# Autodesk Inventor assembly: Ball-Balancing-Robot
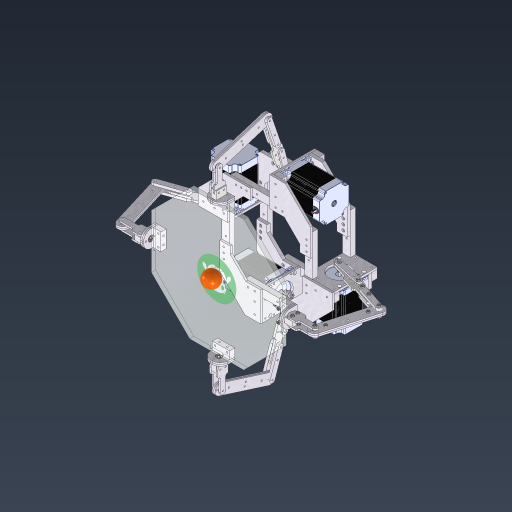
[picture p0: Inventor's stored thumbnail of the model, 512x512]
Saved by Autodesk Inventor 2023 (Build 270158000, 158)
## iProperties
Created: 2024-02-11
Part Number: Ball-Balancing-Robot
Document SubType Name: Assembly
Designer: victo
Author: victo
## Documents named in this file (9)
- C:\Users\victo\Documents\ball-balancing-digital-twin\Mechanics\CAD\Ball-Balancing-Robot.iam
- C:\Users\victo\Documents\ball-balancing-digital-twin\Mechanics\CAD\center_axis.ipt
- C:\Users\victo\Documents\ball-balancing-digital-twin\Mechanics\CAD\MotorArm_3D.iam
- C:\Users\victo\Documents\ball-balancing-digital-twin\Mechanics\CAD\Plate_Acrylic.ipt
- C:\Users\victo\Documents\ball-balancing-digital-twin\Mechanics\CAD\pong_ball.ipt
- C:\Users\victo\OneDrive\Documentos\Inventor\Content Center Files\R2023\en-US\ISO 4762(1)\DIN EN ISO 4762 - M3 x 20.ipt
- C:\Users\victo\OneDrive\Documentos\Inventor\Content Center Files\R2023\en-US\ISO 4762(1)\DIN EN ISO 4762 - M3 x 25.ipt
- C:\Users\victo\OneDrive\Documentos\Inventor\Content Center Files\R2023\en-US\ISO 4762(1)\DIN EN ISO 4762 - M3 x 8.ipt
- C:\Users\victo\OneDrive\Documentos\Inventor\Content Center Files\R2023\en-US\DIN EN ISO 4032\DIN EN ISO 4032 - M3.ipt
## Components (33 placed, 8 different names)
1. center_axis:1
2. MotorArm_3D:1 [sub-assembly] — Mate:1, Mate:2, Flush:1, Angle:1, Mate:9, Mate:10, Mate:11, Mate:34, Mate:35, Mate:36, Mate:37, Mate:38, Mate:39, Mate:40, Mate:41, Mate:42, Mate:43, Mate:44, Mate:45, Mate:46, Mate:47, Mate:48, Mate:49, Mate:50, Mate:51, Mate:52, Mate:53, Mate:54, Mate:56, Mate:61, Mate:63, Mate:65, Mate:68, Mate:69, Mate:71, Mate:73, Mate:75, Mate:77, Mate:78, Mate:79, Mate:80, Mate:81
3. MotorArm_3D:2 [sub-assembly] — Mate:3, Angle:2, Angle:3, Flush:4, Mate:6, Mate:14, Mate:15
4. MotorArm_3D:3 [sub-assembly] — Mate:4, Angle:1, Angle:2, Mate:7, Mate:8, Mate:16, Mate:17
5. MotorArm_3D:4 [sub-assembly] — Mate:5, Angle:3, Flush:2, Flush:3, Mate:12, Mate:13
6. Plate_Acrylic:1 — Mate:9, Mate:10, Mate:11, Mate:12, Mate:13, Mate:14, Mate:15, Mate:16, Mate:17, Tangent:1, Mate:20, Mate:21, Mate:32, Mate:33
7. pong_ball:1 — Tangent:1
8. DIN EN ISO 4762 M3 x 20:3 — Mate:20, Mate:33, Mate:57
9. DIN EN ISO 4762 M3 x 20:4 — Mate:21, Mate:32, Mate:55
10. DIN EN ISO 4762 M3 x 25:4 — Mate:34, Mate:35, Mate:59
11. DIN EN ISO 4762 M3 x 20:5 — Mate:36, Mate:40, Mate:60
12. DIN EN ISO 4762 M3 x 20:6 — Mate:37, Mate:41, Mate:62
13. DIN EN ISO 4762 M3 x 20:7 — Mate:38, Mate:39, Mate:64
14. DIN EN ISO 4762 M3 x 20:8 — Mate:45, Mate:49, Mate:67
15. DIN EN ISO 4762 M3 x 20:9 — Mate:44, Mate:48, Mate:74
16. DIN EN ISO 4762 M3 x 20:10 — Mate:43, Mate:47, Mate:72
17. DIN EN ISO 4762 M3 x 20:11 — Mate:42, Mate:46, Mate:66
18. DIN EN ISO 4762 M3 x 8:1 — Mate:50, Mate:52, Mate:76
19. DIN EN ISO 4762 M3 x 8:2 — Mate:51, Mate:53, Mate:70
20. DIN EN ISO 4032 M3:1 — Mate:56, Mate:57
21. DIN EN ISO 4032 M3:2 — Mate:60, Mate:61
22. DIN EN ISO 4032 M3:3 — Mate:62, Mate:63
23. DIN EN ISO 4032 M3:4 — Mate:59
24. DIN EN ISO 4032 M3:5 — Mate:64, Mate:65
25. DIN EN ISO 4032 M3:6 — Mate:67, Mate:69
26. DIN EN ISO 4032 M3:7 — Mate:66, Mate:68
27. DIN EN ISO 4032 M3:8 — Mate:54, Mate:55
28. DIN EN ISO 4032 M3:9 — Mate:72, Mate:73
29. DIN EN ISO 4032 M3:10 — Mate:74, Mate:75
30. DIN EN ISO 4032 M3:11 — Mate:70, Mate:71
31. DIN EN ISO 4032 M3:12 — Mate:76, Mate:77
32. DIN EN ISO 4762 M3 x 25:5 — Mate:79, Mate:81
33. DIN EN ISO 4762 M3 x 25:6 — Mate:78, Mate:80
## Relationships (76: Mate 68, Flush 4, Angle 3, Tangent 1)
- Mate:1: MotorArm_3D:1
- Mate:2 (71.8 mm): MotorArm_3D:1
- Flush:1 (8.5 mm): MotorArm_3D:1
- Mate:3: MotorArm_3D:2
- Mate:4: MotorArm_3D:3
- Mate:5: MotorArm_3D:4
- Angle:1 (90 deg): MotorArm_3D:1 ↔ MotorArm_3D:3
- Angle:2 (90 deg): MotorArm_3D:2 ↔ MotorArm_3D:3
- Angle:3 (90 deg): MotorArm_3D:2 ↔ MotorArm_3D:4
- Flush:2 (71.8 mm): MotorArm_3D:4
- Flush:3 (8.5 mm): MotorArm_3D:4
- Flush:4 (71.8 mm): MotorArm_3D:2
- Mate:6 (8.5 mm): MotorArm_3D:2
- Mate:7 (71.8 mm): MotorArm_3D:3
- Mate:8 (8.5 mm): MotorArm_3D:3
- Mate:9: MotorArm_3D:1 ↔ Plate_Acrylic:1
- Mate:10: MotorArm_3D:1 ↔ Plate_Acrylic:1
- Mate:11: MotorArm_3D:1 ↔ Plate_Acrylic:1
- Mate:12: MotorArm_3D:4 ↔ Plate_Acrylic:1
- Mate:13: MotorArm_3D:4 ↔ Plate_Acrylic:1
- Mate:14: MotorArm_3D:2 ↔ Plate_Acrylic:1
- Mate:15: MotorArm_3D:2 ↔ Plate_Acrylic:1
- Mate:16: MotorArm_3D:3 ↔ Plate_Acrylic:1
- Mate:17: MotorArm_3D:3 ↔ Plate_Acrylic:1
- Tangent:1: Plate_Acrylic:1 ↔ pong_ball:1
- Mate:20: Plate_Acrylic:1 ↔ DIN EN ISO 4762 M3 x 20:3
- Mate:21: Plate_Acrylic:1 ↔ DIN EN ISO 4762 M3 x 20:4
- Mate:32: Plate_Acrylic:1 ↔ DIN EN ISO 4762 M3 x 20:4
- Mate:33: Plate_Acrylic:1 ↔ DIN EN ISO 4762 M3 x 20:3
- Mate:34: MotorArm_3D:1 ↔ DIN EN ISO 4762 M3 x 25:4
- Mate:35: MotorArm_3D:1 ↔ DIN EN ISO 4762 M3 x 25:4
- Mate:36: MotorArm_3D:1 ↔ DIN EN ISO 4762 M3 x 20:5
- Mate:37: MotorArm_3D:1 ↔ DIN EN ISO 4762 M3 x 20:6
- Mate:38: MotorArm_3D:1 ↔ DIN EN ISO 4762 M3 x 20:7
- Mate:39: MotorArm_3D:1 ↔ DIN EN ISO 4762 M3 x 20:7
- Mate:40: MotorArm_3D:1 ↔ DIN EN ISO 4762 M3 x 20:5
- Mate:41: MotorArm_3D:1 ↔ DIN EN ISO 4762 M3 x 20:6
- Mate:42: MotorArm_3D:1 ↔ DIN EN ISO 4762 M3 x 20:11
- Mate:43: MotorArm_3D:1 ↔ DIN EN ISO 4762 M3 x 20:10
- Mate:44: MotorArm_3D:1 ↔ DIN EN ISO 4762 M3 x 20:9
- Mate:45: MotorArm_3D:1 ↔ DIN EN ISO 4762 M3 x 20:8
- Mate:46: MotorArm_3D:1 ↔ DIN EN ISO 4762 M3 x 20:11
- Mate:47: MotorArm_3D:1 ↔ DIN EN ISO 4762 M3 x 20:10
- Mate:48: MotorArm_3D:1 ↔ DIN EN ISO 4762 M3 x 20:9
- Mate:49: MotorArm_3D:1 ↔ DIN EN ISO 4762 M3 x 20:8
- Mate:50: MotorArm_3D:1 ↔ DIN EN ISO 4762 M3 x 8:1
- Mate:51: MotorArm_3D:1 ↔ DIN EN ISO 4762 M3 x 8:2
- Mate:52: MotorArm_3D:1 ↔ DIN EN ISO 4762 M3 x 8:1
- Mate:53: MotorArm_3D:1 ↔ DIN EN ISO 4762 M3 x 8:2
- Mate:54: MotorArm_3D:1 ↔ DIN EN ISO 4032 M3:8
- Mate:55: DIN EN ISO 4762 M3 x 20:4 ↔ DIN EN ISO 4032 M3:8
- Mate:56: MotorArm_3D:1 ↔ DIN EN ISO 4032 M3:1
- Mate:57: DIN EN ISO 4762 M3 x 20:3 ↔ DIN EN ISO 4032 M3:1
- Mate:59: DIN EN ISO 4762 M3 x 25:4 ↔ DIN EN ISO 4032 M3:4
- Mate:60: DIN EN ISO 4762 M3 x 20:5 ↔ DIN EN ISO 4032 M3:2
- Mate:61: MotorArm_3D:1 ↔ DIN EN ISO 4032 M3:2
- Mate:62: DIN EN ISO 4762 M3 x 20:6 ↔ DIN EN ISO 4032 M3:3
- Mate:63: MotorArm_3D:1 ↔ DIN EN ISO 4032 M3:3
- Mate:64: DIN EN ISO 4762 M3 x 20:7 ↔ DIN EN ISO 4032 M3:5
- Mate:65: MotorArm_3D:1 ↔ DIN EN ISO 4032 M3:5
- Mate:66: DIN EN ISO 4762 M3 x 20:11 ↔ DIN EN ISO 4032 M3:7
- Mate:67: DIN EN ISO 4762 M3 x 20:8 ↔ DIN EN ISO 4032 M3:6
- Mate:68: MotorArm_3D:1 ↔ DIN EN ISO 4032 M3:7
- Mate:69: MotorArm_3D:1 ↔ DIN EN ISO 4032 M3:6
- Mate:70: DIN EN ISO 4762 M3 x 8:2 ↔ DIN EN ISO 4032 M3:11
- Mate:71: MotorArm_3D:1 ↔ DIN EN ISO 4032 M3:11
- Mate:72: DIN EN ISO 4762 M3 x 20:10 ↔ DIN EN ISO 4032 M3:9
- Mate:73: MotorArm_3D:1 ↔ DIN EN ISO 4032 M3:9
- Mate:74: DIN EN ISO 4762 M3 x 20:9 ↔ DIN EN ISO 4032 M3:10
- Mate:75: MotorArm_3D:1 ↔ DIN EN ISO 4032 M3:10
- Mate:76: DIN EN ISO 4762 M3 x 8:1 ↔ DIN EN ISO 4032 M3:12
- Mate:77: MotorArm_3D:1 ↔ DIN EN ISO 4032 M3:12
- Mate:78: MotorArm_3D:1 ↔ DIN EN ISO 4762 M3 x 25:6
- Mate:79: MotorArm_3D:1 ↔ DIN EN ISO 4762 M3 x 25:5
- Mate:80: MotorArm_3D:1 ↔ DIN EN ISO 4762 M3 x 25:6
- Mate:81: MotorArm_3D:1 ↔ DIN EN ISO 4762 M3 x 25:5
